# Autodesk Inventor assembly: field_and_shooter
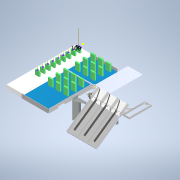
[picture p0: Inventor's stored thumbnail of the model, 180x180]
Saved by Autodesk Inventor 2022 (Build 260153000, 153)
## iProperties
Created: 2021-09-13
Part Number: field_and_shooter
Document SubType Name: Assembly
Designer: yuto6
Author: yuto6
## Documents named in this file (18)
- C:\Users\yuto6\Box\Public_Share\キャチロボバトルコンテスト2021\CAD\catchrobo_hardware\assy-shooter\field_and_shooter.iam
- C:\Users\yuto6\Box\Public_Share\キャチロボバトルコンテスト2021\CAD\catchrobo_hardware\field\aassy-blue_side.iam
- C:\Users\yuto6\Box\Public_Share\キャチロボバトルコンテスト2021\CAD\catchrobo_hardware\assy-shooter\s-assy-shooter_frame.iam
- C:\Users\yuto6\Box\Public_Share\キャチロボバトルコンテスト2021\CAD\catchrobo_hardware\assy-shooter\s-assy-shooter_unit.iam
- C:\Users\yuto6\Box\Public_Share\キャチロボバトルコンテスト2021\CAD\catchrobo_hardware\assy-shooter\s_carbon_plate1.ipt
- C:\Users\yuto6\Box\Public_Share\キャチロボバトルコンテスト2021\CAD\catchrobo_hardware\assy-shooter\s_base2.ipt
- C:\Users\yuto6\Box\Public_Share\キャチロボバトルコンテスト2021\CAD\catchrobo_hardware\assy-shooter\s-assy-sorter.iam
- C:\Users\yuto6\Box\Public_Share\キャチロボバトルコンテスト2021\CAD\catchrobo_hardware\assy-shooter\s_base4_2.ipt
- C:\Users\yuto6\Box\Public_Share\キャチロボバトルコンテスト2021\CAD\catchrobo_hardware\assy-shooter\SCSTR6-8.iam
- C:\Users\yuto6\Box\Public_Share\キャチロボバトルコンテスト2021\CAD\catchrobo_hardware\assy-shooter\s_carbon_plate5.ipt
- C:\Users\yuto6\Box\Public_Share\キャチロボバトルコンテスト2021\CAD\catchrobo_hardware\assy-shooter\s-assy-frame-connector.iam
- C:\Users\yuto6\Box\Public_Share\キャチロボバトルコンテスト2021\CAD\catchrobo_hardware\assy-shooter\MF126ZZ.iam
- C:\Users\yuto6\Box\Public_Share\キャチロボバトルコンテスト2021\CAD\catchrobo_hardware\assy-shooter\CBSTSR3-5.ipt
- C:\Users\yuto6\Box\Public_Share\キャチロボバトルコンテスト2021\CAD\catchrobo_hardware\assy-shooter\CBSTSR3-10.ipt
- C:\Users\yuto6\Box\Public_Share\キャチロボバトルコンテスト2021\CAD\catchrobo_hardware\assy-shooter\HNT3-ST-M3_214.ipt
- C:\Users\yuto6\Box\Public_Share\キャチロボバトルコンテスト2021\CAD\catchrobo_hardware\assy-shooter\s-assy-waight_holder.iam
- C:\Users\yuto6\Box\Public_Share\キャチロボバトルコンテスト2021\CAD\catchrobo_hardware\assy-shooter\CB3-6.ipt
- C:\Users\yuto6\Box\Public_Share\キャチロボバトルコンテスト2021\CAD\catchrobo_hardware\assy-shooter\CBSTSE4-10.ipt
## Components (75 placed, 17 different names)
1. aassy-blue_side:1 [sub-assembly] — メイト:1, フラッシュ:1, フラッシュ:2, フラッシュ:3, メイト:2
2. s-assy-shooter_frame:1 [sub-assembly] — メイト:1, フラッシュ:1, フラッシュ:41, メイト:39, フラッシュ:42, メイト:41, フラッシュ:43, メイト:43, フラッシュ:44, メイト:45, フラッシュ:45, メイト:125
3. s-assy-shooter_unit:1 [sub-assembly] — フラッシュ:2, フラッシュ:3, メイト:2, メイト:5, フラッシュ:5, メイト:6, メイト:25, メイト:26, メイト:27, フラッシュ:40, メイト:40, メイト:42, メイト:53, メイト:54, メイト:55, メイト:56, メイト:57, メイト:58, メイト:59, メイト:60, メイト:93, メイト:94, メイト:95, メイト:96, メイト:97, メイト:98, メイト:99, メイト:100, メイト:114, メイト:116, メイト:118, メイト:120, メイト:122, メイト:124, メイト:141, メイト:142, メイト:143, メイト:146, メイト:147, メイト:148, メイト:149, メイト:150, メイト:151, メイト:152, メイト:153, メイト:162, メイト:163, メイト:164
4. s_carbon_plate1:1 — メイト:5, フラッシュ:5, メイト:6, メイト:7, フラッシュ:6, メイト:8, メイト:11, メイト:12, メイト:13, メイト:61, メイト:62, メイト:63, メイト:64, メイト:65, メイト:66, メイト:67, メイト:68, メイト:85, メイト:86, メイト:87, メイト:88, メイト:89, メイト:90, メイト:91, メイト:92
5. s_carbon_plate1:2 — メイト:9, フラッシュ:7, メイト:10, メイト:21, フラッシュ:11, メイト:22, メイト:36, メイト:37, メイト:38, メイト:46, メイト:69, メイト:70, メイト:71, メイト:72, メイト:73, メイト:74, メイト:75, メイト:76, メイト:77, メイト:78, メイト:79, メイト:80, メイト:81, メイト:82, メイト:83, メイト:84, メイト:154, メイト:155, メイト:156, メイト:157, メイト:158, メイト:159, メイト:160, メイト:161
6. s_base2:1 — メイト:7, フラッシュ:6, メイト:8, メイト:9, フラッシュ:7, メイト:10, メイト:44, メイト:47, メイト:48, メイト:49, メイト:50, メイト:107, メイト:108, メイト:110, メイト:112
7. s-assy-sorter:1 [sub-assembly] — メイト:11, メイト:12, メイト:13
8. s_base4_2:1 — メイト:21, フラッシュ:11, メイト:22, メイト:51, メイト:52, メイト:102, メイト:104, メイト:144, メイト:145
9. SCSTR6-8:1 [sub-assembly] — メイト:25, メイト:26, メイト:28, メイト:29, メイト:31, メイト:32, メイト:126, メイト:128, メイト:130
10. SCSTR6-8:2 [sub-assembly] — メイト:27, メイト:28, メイト:33, メイト:34, メイト:35, メイト:132, メイト:134, メイト:136
11. s_carbon_plate5:1 — メイト:29, メイト:31, メイト:32, フラッシュ:40, フラッシュ:14, メイト:127, メイト:129, メイト:131
12. s_carbon_plate5:2 — メイト:33, メイト:34, メイト:35, フラッシュ:14, メイト:133, メイト:135, メイト:137
13. s-assy-sorter:2 [sub-assembly] — メイト:36, メイト:37, メイト:38
14. s-assy-frame-connector:1 [sub-assembly] — フラッシュ:41, メイト:39, メイト:40
15. s-assy-frame-connector:2 [sub-assembly] — フラッシュ:42, メイト:41, メイト:42
16. s-assy-frame-connector:3 [sub-assembly] — フラッシュ:43, メイト:43, メイト:44
17. s-assy-frame-connector:4 [sub-assembly] — フラッシュ:44, メイト:45, メイト:46
18. MF126ZZ:1 [sub-assembly] — メイト:49, メイト:50
19. MF126ZZ:2 [sub-assembly] — メイト:51, メイト:52
20. MF126ZZ:3 [sub-assembly] — メイト:47, メイト:48
21. CBSTSR3-5:1 — メイト:67, メイト:68
22. CBSTSR3-5:2 — メイト:63, メイト:64
23. CBSTSR3-5:3 — メイト:65, メイト:66
24. CBSTSR3-5:4 — メイト:61, メイト:62
25. CBSTSR3-5:5 — メイト:53, メイト:54
26. CBSTSR3-5:6 — メイト:59, メイト:60
27. CBSTSR3-5:7 — メイト:57, メイト:58
28. CBSTSR3-5:8 — メイト:55, メイト:56
29. CBSTSR3-5:9 — メイト:71, メイト:72
30. CBSTSR3-5:10 — メイト:73, メイト:74
31. CBSTSR3-5:11 — メイト:75, メイト:76
32. CBSTSR3-5:12 — メイト:69, メイト:70
33. CBSTSR3-10:1 — メイト:81, メイト:82, メイト:106
34. CBSTSR3-10:2 — メイト:87, メイト:88, メイト:111
35. CBSTSR3-10:3 — メイト:83, メイト:84, メイト:105
36. CBSTSR3-10:4 — メイト:85, メイト:86, メイト:109
37. CBSTSR3-10:5 — メイト:89, メイト:90, メイト:115
38. CBSTSR3-10:6 — メイト:91, メイト:92, メイト:113
39. CBSTSR3-10:7 — メイト:93, メイト:94, メイト:119
40. CBSTSR3-10:8 — メイト:95, メイト:96, メイト:117
41. CBSTSR3-10:9 — メイト:77, メイト:78, メイト:103
42. CBSTSR3-10:10 — メイト:79, メイト:80, メイト:101
43. CBSTSR3-10:11 — メイト:97, メイト:98, メイト:123
44. CBSTSR3-10:12 — メイト:99, メイト:100, メイト:121
45. HNT3-ST-M3_214:1 — メイト:113, メイト:114
46. HNT3-ST-M3_214:2 — メイト:115, メイト:116
47. HNT3-ST-M3_214:3 — メイト:121, メイト:122
48. HNT3-ST-M3_214:4 — メイト:103, メイト:104
49. HNT3-ST-M3_214:5 — メイト:111, メイト:112
50. HNT3-ST-M3_214:6 — メイト:117, メイト:118
51. HNT3-ST-M3_214:7 — メイト:105, メイト:108
52. HNT3-ST-M3_214:8 — メイト:101, メイト:102
53. HNT3-ST-M3_214:9 — メイト:119, メイト:120
54. HNT3-ST-M3_214:10 — メイト:123, メイト:124
55. HNT3-ST-M3_214:11 — メイト:109, メイト:110
56. HNT3-ST-M3_214:12 — メイト:106, メイト:107
57. s-assy-waight_holder:1 [sub-assembly] — フラッシュ:45, メイト:125
58. CB3-6:1 — メイト:134, メイト:135
59. CB3-6:2 — メイト:130, メイト:131
60. CB3-6:3 — メイト:132, メイト:133
61. CB3-6:4 — メイト:126, メイト:127
62. CB3-6:5 — メイト:128, メイト:129
63. CB3-6:7 — メイト:136, メイト:137
64. CBSTSE4-10:1 — メイト:141, メイト:164
65. CBSTSE4-10:2 — メイト:142, メイト:162
66. CBSTSE4-10:3 — メイト:143, メイト:163
67. MF126ZZ:4 [sub-assembly] — メイト:144, メイト:145
68. CBSTSR3-10:13 — メイト:155, メイト:157
69. CBSTSR3-10:14 — メイト:146, メイト:152
70. CBSTSR3-10:15 — メイト:149, メイト:151
71. CBSTSR3-10:17 — メイト:158, メイト:160
72. CBSTSR3-10:18 — メイト:159, メイト:161
73. CBSTSR3-10:22 — メイト:154, メイト:156
74. CBSTSR3-10:23 — メイト:148, メイト:150
75. CBSTSR3-10:24 — メイト:147, メイト:153
## Relationships (163: Mate 149, Flush 14)
- メイト:1 [Mate]: aassy-blue_side:1 ↔ s-assy-shooter_frame:1
- フラッシュ:1 [Flush] (60 mm): aassy-blue_side:1 ↔ s-assy-shooter_frame:1
- フラッシュ:2 [Flush]: aassy-blue_side:1 ↔ s-assy-shooter_unit:1
- フラッシュ:3 [Flush]: aassy-blue_side:1 ↔ s-assy-shooter_unit:1
- メイト:2 [Mate] (2 mm): aassy-blue_side:1 ↔ s-assy-shooter_unit:1
- メイト:5 [Mate]: s-assy-shooter_unit:1 ↔ s_carbon_plate1:1
- フラッシュ:5 [Flush]: s-assy-shooter_unit:1 ↔ s_carbon_plate1:1
- メイト:6 [Mate]: s-assy-shooter_unit:1 ↔ s_carbon_plate1:1
- メイト:7 [Mate]: s_carbon_plate1:1 ↔ s_base2:1
- フラッシュ:6 [Flush]: s_carbon_plate1:1 ↔ s_base2:1
- メイト:8 [Mate]: s_carbon_plate1:1 ↔ s_base2:1
- メイト:9 [Mate]: s_carbon_plate1:2 ↔ s_base2:1
- フラッシュ:7 [Flush]: s_carbon_plate1:2 ↔ s_base2:1
- メイト:10 [Mate]: s_carbon_plate1:2 ↔ s_base2:1
- メイト:11 [Mate]: s_carbon_plate1:1 ↔ s-assy-sorter:1
- メイト:12 [Mate]: s_carbon_plate1:1 ↔ s-assy-sorter:1
- メイト:13 [Mate]: s_carbon_plate1:1 ↔ s-assy-sorter:1
- メイト:21 [Mate]: s_carbon_plate1:2 ↔ s_base4_2:1
- フラッシュ:11 [Flush]: s_carbon_plate1:2 ↔ s_base4_2:1
- メイト:22 [Mate]: s_carbon_plate1:2 ↔ s_base4_2:1
- メイト:25 [Mate]: s-assy-shooter_unit:1 ↔ SCSTR6-8:1
- メイト:26 [Mate] (195 mm): s-assy-shooter_unit:1 ↔ SCSTR6-8:1
- メイト:27 [Mate]: s-assy-shooter_unit:1 ↔ SCSTR6-8:2
- メイト:28 [Mate] (195 mm): SCSTR6-8:1 ↔ SCSTR6-8:2
- メイト:29 [Mate]: SCSTR6-8:1 ↔ s_carbon_plate5:1
- メイト:31 [Mate]: SCSTR6-8:1 ↔ s_carbon_plate5:1
- メイト:32 [Mate]: SCSTR6-8:1 ↔ s_carbon_plate5:1
- メイト:33 [Mate]: SCSTR6-8:2 ↔ s_carbon_plate5:2
- メイト:34 [Mate]: SCSTR6-8:2 ↔ s_carbon_plate5:2
- メイト:35 [Mate]: SCSTR6-8:2 ↔ s_carbon_plate5:2
- メイト:36 [Mate]: s_carbon_plate1:2 ↔ s-assy-sorter:2
- メイト:37 [Mate]: s_carbon_plate1:2 ↔ s-assy-sorter:2
- メイト:38 [Mate]: s_carbon_plate1:2 ↔ s-assy-sorter:2
- フラッシュ:40 [Flush]: s-assy-shooter_unit:1 ↔ s_carbon_plate5:1
- フラッシュ:14 [Flush]: s_carbon_plate5:1 ↔ s_carbon_plate5:2
- フラッシュ:41 [Flush]: s-assy-shooter_frame:1 ↔ s-assy-frame-connector:1
- メイト:39 [Mate]: s-assy-shooter_frame:1 ↔ s-assy-frame-connector:1
- メイト:40 [Mate]: s-assy-shooter_unit:1 ↔ s-assy-frame-connector:1
- フラッシュ:42 [Flush]: s-assy-shooter_frame:1 ↔ s-assy-frame-connector:2
- メイト:41 [Mate]: s-assy-shooter_frame:1 ↔ s-assy-frame-connector:2
- メイト:42 [Mate]: s-assy-shooter_unit:1 ↔ s-assy-frame-connector:2
- フラッシュ:43 [Flush]: s-assy-shooter_frame:1 ↔ s-assy-frame-connector:3
- メイト:43 [Mate]: s-assy-shooter_frame:1 ↔ s-assy-frame-connector:3
- メイト:44 [Mate]: s_base2:1 ↔ s-assy-frame-connector:3
- フラッシュ:44 [Flush]: s-assy-shooter_frame:1 ↔ s-assy-frame-connector:4
- メイト:45 [Mate]: s-assy-shooter_frame:1 ↔ s-assy-frame-connector:4
- メイト:46 [Mate]: s_carbon_plate1:2 ↔ s-assy-frame-connector:4
- メイト:47 [Mate]: s_base2:1 ↔ MF126ZZ:3
- メイト:48 [Mate]: s_base2:1 ↔ MF126ZZ:3
- メイト:49 [Mate]: s_base2:1 ↔ MF126ZZ:1
- メイト:50 [Mate]: s_base2:1 ↔ MF126ZZ:1
- メイト:51 [Mate]: s_base4_2:1 ↔ MF126ZZ:2
- メイト:52 [Mate]: s_base4_2:1 ↔ MF126ZZ:2
- メイト:53 [Mate]: s-assy-shooter_unit:1 ↔ CBSTSR3-5:5
- メイト:54 [Mate]: s-assy-shooter_unit:1 ↔ CBSTSR3-5:5
- メイト:55 [Mate]: s-assy-shooter_unit:1 ↔ CBSTSR3-5:8
- メイト:56 [Mate]: s-assy-shooter_unit:1 ↔ CBSTSR3-5:8
- メイト:57 [Mate]: s-assy-shooter_unit:1 ↔ CBSTSR3-5:7
- メイト:58 [Mate]: s-assy-shooter_unit:1 ↔ CBSTSR3-5:7
- メイト:59 [Mate]: s-assy-shooter_unit:1 ↔ CBSTSR3-5:6
- メイト:60 [Mate]: s-assy-shooter_unit:1 ↔ CBSTSR3-5:6
- メイト:61 [Mate]: s_carbon_plate1:1 ↔ CBSTSR3-5:4
- メイト:62 [Mate]: s_carbon_plate1:1 ↔ CBSTSR3-5:4
- メイト:63 [Mate]: s_carbon_plate1:1 ↔ CBSTSR3-5:2
- メイト:64 [Mate]: s_carbon_plate1:1 ↔ CBSTSR3-5:2
- メイト:65 [Mate]: s_carbon_plate1:1 ↔ CBSTSR3-5:3
- メイト:66 [Mate]: s_carbon_plate1:1 ↔ CBSTSR3-5:3
- メイト:67 [Mate]: s_carbon_plate1:1 ↔ CBSTSR3-5:1
- メイト:68 [Mate]: s_carbon_plate1:1 ↔ CBSTSR3-5:1
- メイト:69 [Mate]: s_carbon_plate1:2 ↔ CBSTSR3-5:12
- メイト:70 [Mate]: s_carbon_plate1:2 ↔ CBSTSR3-5:12
- メイト:71 [Mate]: s_carbon_plate1:2 ↔ CBSTSR3-5:9
- メイト:72 [Mate]: s_carbon_plate1:2 ↔ CBSTSR3-5:9
- メイト:73 [Mate]: s_carbon_plate1:2 ↔ CBSTSR3-5:10
- メイト:74 [Mate]: s_carbon_plate1:2 ↔ CBSTSR3-5:10
- メイト:75 [Mate]: s_carbon_plate1:2 ↔ CBSTSR3-5:11
- メイト:76 [Mate]: s_carbon_plate1:2 ↔ CBSTSR3-5:11
- メイト:77 [Mate]: s_carbon_plate1:2 ↔ CBSTSR3-10:9
- メイト:78 [Mate]: s_carbon_plate1:2 ↔ CBSTSR3-10:9
- メイト:79 [Mate]: s_carbon_plate1:2 ↔ CBSTSR3-10:10
- メイト:80 [Mate]: s_carbon_plate1:2 ↔ CBSTSR3-10:10
- メイト:81 [Mate]: s_carbon_plate1:2 ↔ CBSTSR3-10:1
- メイト:82 [Mate]: s_carbon_plate1:2 ↔ CBSTSR3-10:1
- メイト:83 [Mate]: s_carbon_plate1:2 ↔ CBSTSR3-10:3
- メイト:84 [Mate]: s_carbon_plate1:2 ↔ CBSTSR3-10:3
- メイト:85 [Mate]: s_carbon_plate1:1 ↔ CBSTSR3-10:4
- メイト:86 [Mate]: s_carbon_plate1:1 ↔ CBSTSR3-10:4
- メイト:87 [Mate]: s_carbon_plate1:1 ↔ CBSTSR3-10:2
- メイト:88 [Mate]: s_carbon_plate1:1 ↔ CBSTSR3-10:2
- メイト:89 [Mate]: s_carbon_plate1:1 ↔ CBSTSR3-10:5
- メイト:90 [Mate]: s_carbon_plate1:1 ↔ CBSTSR3-10:5
- メイト:91 [Mate]: s_carbon_plate1:1 ↔ CBSTSR3-10:6
- メイト:92 [Mate]: s_carbon_plate1:1 ↔ CBSTSR3-10:6
- メイト:93 [Mate]: s-assy-shooter_unit:1 ↔ CBSTSR3-10:7
- メイト:94 [Mate]: s-assy-shooter_unit:1 ↔ CBSTSR3-10:7
- メイト:95 [Mate]: s-assy-shooter_unit:1 ↔ CBSTSR3-10:8
- メイト:96 [Mate]: s-assy-shooter_unit:1 ↔ CBSTSR3-10:8
- メイト:97 [Mate]: s-assy-shooter_unit:1 ↔ CBSTSR3-10:11
- メイト:98 [Mate]: s-assy-shooter_unit:1 ↔ CBSTSR3-10:11
- メイト:99 [Mate]: s-assy-shooter_unit:1 ↔ CBSTSR3-10:12
- メイト:100 [Mate]: s-assy-shooter_unit:1 ↔ CBSTSR3-10:12
- メイト:101 [Mate]: CBSTSR3-10:10 ↔ HNT3-ST-M3_214:8
- メイト:102 [Mate]: s_base4_2:1 ↔ HNT3-ST-M3_214:8
- メイト:103 [Mate]: CBSTSR3-10:9 ↔ HNT3-ST-M3_214:4
- メイト:104 [Mate]: s_base4_2:1 ↔ HNT3-ST-M3_214:4
- メイト:105 [Mate]: CBSTSR3-10:3 ↔ HNT3-ST-M3_214:7
- メイト:106 [Mate]: CBSTSR3-10:1 ↔ HNT3-ST-M3_214:12
- メイト:107 [Mate]: s_base2:1 ↔ HNT3-ST-M3_214:12
- メイト:108 [Mate]: s_base2:1 ↔ HNT3-ST-M3_214:7
- メイト:109 [Mate]: CBSTSR3-10:4 ↔ HNT3-ST-M3_214:11
- メイト:110 [Mate]: s_base2:1 ↔ HNT3-ST-M3_214:11
- メイト:111 [Mate]: CBSTSR3-10:2 ↔ HNT3-ST-M3_214:5
- メイト:112 [Mate]: s_base2:1 ↔ HNT3-ST-M3_214:5
- メイト:113 [Mate]: CBSTSR3-10:6 ↔ HNT3-ST-M3_214:1
- メイト:114 [Mate]: s-assy-shooter_unit:1 ↔ HNT3-ST-M3_214:1
- メイト:115 [Mate]: CBSTSR3-10:5 ↔ HNT3-ST-M3_214:2
- メイト:116 [Mate]: s-assy-shooter_unit:1 ↔ HNT3-ST-M3_214:2
- メイト:117 [Mate]: CBSTSR3-10:8 ↔ HNT3-ST-M3_214:6
- メイト:118 [Mate]: s-assy-shooter_unit:1 ↔ HNT3-ST-M3_214:6
- メイト:119 [Mate]: CBSTSR3-10:7 ↔ HNT3-ST-M3_214:9
- メイト:120 [Mate]: s-assy-shooter_unit:1 ↔ HNT3-ST-M3_214:9
- メイト:121 [Mate]: CBSTSR3-10:12 ↔ HNT3-ST-M3_214:3
- メイト:122 [Mate]: s-assy-shooter_unit:1 ↔ HNT3-ST-M3_214:3
- メイト:123 [Mate]: CBSTSR3-10:11 ↔ HNT3-ST-M3_214:10
- メイト:124 [Mate]: s-assy-shooter_unit:1 ↔ HNT3-ST-M3_214:10
- フラッシュ:45 [Flush]: s-assy-shooter_frame:1 ↔ s-assy-waight_holder:1
- メイト:125 [Mate]: s-assy-shooter_frame:1 ↔ s-assy-waight_holder:1
- メイト:126 [Mate]: SCSTR6-8:1 ↔ CB3-6:4
- メイト:127 [Mate]: s_carbon_plate5:1 ↔ CB3-6:4
- メイト:128 [Mate]: SCSTR6-8:1 ↔ CB3-6:5
- メイト:129 [Mate]: s_carbon_plate5:1 ↔ CB3-6:5
- メイト:130 [Mate]: SCSTR6-8:1 ↔ CB3-6:2
- メイト:131 [Mate]: s_carbon_plate5:1 ↔ CB3-6:2
- メイト:132 [Mate]: SCSTR6-8:2 ↔ CB3-6:3
- メイト:133 [Mate]: s_carbon_plate5:2 ↔ CB3-6:3
- メイト:134 [Mate]: SCSTR6-8:2 ↔ CB3-6:1
- メイト:135 [Mate]: s_carbon_plate5:2 ↔ CB3-6:1
- メイト:136 [Mate]: SCSTR6-8:2 ↔ CB3-6:7
- メイト:137 [Mate]: s_carbon_plate5:2 ↔ CB3-6:7
- メイト:141 [Mate]: s-assy-shooter_unit:1 ↔ CBSTSE4-10:1
- メイト:142 [Mate]: s-assy-shooter_unit:1 ↔ CBSTSE4-10:2
- メイト:143 [Mate]: s-assy-shooter_unit:1 ↔ CBSTSE4-10:3
- メイト:144 [Mate]: s_base4_2:1 ↔ MF126ZZ:4
- メイト:145 [Mate]: s_base4_2:1 ↔ MF126ZZ:4
- メイト:146 [Mate]: s-assy-shooter_unit:1 ↔ CBSTSR3-10:14
- メイト:147 [Mate]: s-assy-shooter_unit:1 ↔ CBSTSR3-10:24
- メイト:148 [Mate]: s-assy-shooter_unit:1 ↔ CBSTSR3-10:23
- メイト:149 [Mate]: s-assy-shooter_unit:1 ↔ CBSTSR3-10:15
- メイト:150 [Mate]: s-assy-shooter_unit:1 ↔ CBSTSR3-10:23
- メイト:151 [Mate]: s-assy-shooter_unit:1 ↔ CBSTSR3-10:15
- メイト:152 [Mate]: s-assy-shooter_unit:1 ↔ CBSTSR3-10:14
- メイト:153 [Mate]: s-assy-shooter_unit:1 ↔ CBSTSR3-10:24
- メイト:154 [Mate]: s_carbon_plate1:2 ↔ CBSTSR3-10:22
- メイト:155 [Mate]: s_carbon_plate1:2 ↔ CBSTSR3-10:13
- メイト:156 [Mate]: s_carbon_plate1:2 ↔ CBSTSR3-10:22
- メイト:157 [Mate]: s_carbon_plate1:2 ↔ CBSTSR3-10:13
- メイト:158 [Mate]: s_carbon_plate1:2 ↔ CBSTSR3-10:17
- メイト:159 [Mate]: s_carbon_plate1:2 ↔ CBSTSR3-10:18
- メイト:160 [Mate]: s_carbon_plate1:2 ↔ CBSTSR3-10:17
- メイト:161 [Mate]: s_carbon_plate1:2 ↔ CBSTSR3-10:18
- メイト:162 [Mate]: s-assy-shooter_unit:1 ↔ CBSTSE4-10:2
- メイト:163 [Mate]: s-assy-shooter_unit:1 ↔ CBSTSE4-10:3
- メイト:164 [Mate]: s-assy-shooter_unit:1 ↔ CBSTSE4-10:1
